# Autodesk Inventor assembly: TEcahing
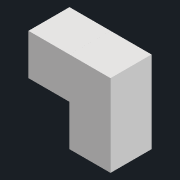
[picture p0: Inventor's stored thumbnail of the model, 180x180]
Saved by Autodesk Inventor 2022 (Build 260153000, 153)
## iProperties
Created: 2021-09-17
Part Number: TEcahing
Document SubType Name: Assembly
Designer: divid
Author: divid
## Documents named in this file (2)
- C:\Users\divid\Documents\GitHub\ComputerAidedDesign\2021-22\FTC\#13822 Robovikes\TEcahing.iam
- C:\Users\divid\Documents\GitHub\ComputerAidedDesign\2021-22\FTC\#13822 Robovikes\TEaching.ipt
## Components (3 placed, 1 different names)
1. TEaching:1 — Mate:1, Flush:1, Flush:2, Mate:2, Flush:3, Mate:3, Flush:4
2. TEaching:2 — Mate:2, Flush:3, Mate:3, Flush:4
3. TEaching:3 — Mate:1, Flush:1, Flush:2
## Relationships (7: Flush 4, Mate 3)
- Mate:1: TEaching:1 ↔ TEaching:3
- Flush:1: TEaching:1 ↔ TEaching:3
- Flush:2: TEaching:1 ↔ TEaching:3
- Mate:2: TEaching:1 ↔ TEaching:2
- Flush:3: TEaching:1 ↔ TEaching:2
- Mate:3: TEaching:1 ↔ TEaching:2
- Flush:4: TEaching:1 ↔ TEaching:2
